# Autodesk Inventor assembly: Hand
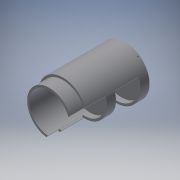
[picture p0: Inventor's stored thumbnail of the model, 180x180]
Saved by Autodesk Inventor 2016 (Build 200138000, 138)
## iProperties
Created: 2016-11-10
Part Number: Hand
Material: 一般
Document SubType Name: Assembly
Designer: Daisuke
Author: Daisuke
## Documents named in this file (3)
- C:\Users\Daisuke\Documents\GitHub\CAD\Hand\ver1\Hand.iam
- C:\Users\Daisuke\Documents\GitHub\CAD\Hand\ver1\insideHand.iam
- C:\Users\Daisuke\Documents\GitHub\CAD\Hand\ver1\outsideHand.iam
## Components (2 placed, 2 different names)
1. insideHand:1 [sub-assembly] — 挿入:1
2. outsideHand:1 [sub-assembly] — 挿入:1
## Relationships (1: Insert 1)
- 挿入:1 [Insert]: insideHand:1 ↔ outsideHand:1
